# Autodesk Inventor assembly: pld-assembly
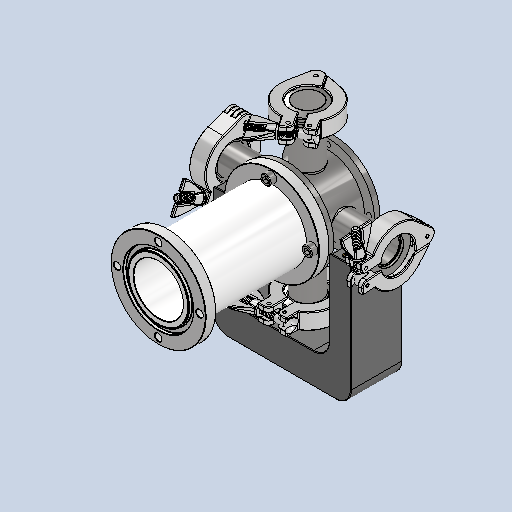
[picture p0: Inventor's stored thumbnail of the model, 512x512]
Saved by Autodesk Inventor 2026 (Build 300175050, 175E)
## iProperties
Created: 2025-11-13
Part Number: pld-assembly
Document SubType Name: Assembly
Designer: kuzmin
Author: kuzmin
## Documents named in this file (12)
- C:\Users\queez\Dropbox\Drawings\PIHTI\PLD\pld-assembly.iam
- C:\Users\queez\Dropbox\Drawings\PIHTI\PLD\pld-vessel-gasket.ipt
- C:\Users\queez\Dropbox\Drawings\PIHTI\ContentCenter\NW\NW25_clamp.ipt
- C:\Users\queez\Dropbox\Drawings\PIHTI\PLD\pld-vessel.iam
- C:\Users\queez\Dropbox\Drawings\PIHTI\PLD\pld_nipple.iam
- C:\Users\queez\Dropbox\Drawings\PIHTI\ContentCenter\Fastners\M6x16-SHCS.ipt
- C:\Users\queez\Dropbox\Drawings\PIHTI\PLD\pld-support.ipt
- C:\Users\queez\Dropbox\Drawings\PIHTI\ContentCenter\Fastners\brass-insert-m3x5.ipt
- C:\Users\queez\Dropbox\Drawings\PIHTI\ContentCenter\NW\NW25-blank.ipt
- C:\Users\queez\Dropbox\Drawings\PIHTI\PLD\pld-sample-holder.ipt
- C:\Users\queez\Dropbox\Drawings\PIHTI\PLD\m4x60-pin.ipt
- C:\Users\queez\Dropbox\Drawings\PIHTI\PLD\pld-target-holder.ipt
## Components (21 placed, 11 different names)
1. pld-vessel:1 [sub-assembly] — Rigid:7, Mate:2, Mate:3, Flush:2, Mate:5, Mate:6, Mate:7, Flush:3, Mate:8, Mate:9, Rigid:16, Rigid:18, Flush:4
2. pld-vessel-gasket:1
3. pld-vessel-gasket:2
4. NW25_clamp:1
5. pld_nipple:1 [sub-assembly] — Rigid:7, Rigid:8, Rigid:9, Rigid:10, Rigid:11
6. pld-support:1 — Mate:2, Mate:4, Rigid:12, Rigid:13, Rigid:14, Rigid:15, Mate:10
7. NW25_clamp:2 — Mate:5, Flush:3
8. NW25_clamp:3 — Mate:6, Mate:8
9. NW25_clamp:4 — Mate:7, Mate:9
10. brass-insert-m3x5:1 — Rigid:14
11. brass-insert-m3x5:2 — Rigid:13
12. brass-insert-m3x5:3 — Rigid:15
13. brass-insert-m3x5:4 — Rigid:12
14. NW25-blank:1 — Rigid:16, Rigid:17
15. pld-sample-holder:1 — Rotational:1
16. m4x60-pin:1 — Rigid:17, Rotational:1
17. pld-target-holder:1 — Rigid:18
18. JIS B 1176 - Metric M6 x 16:1 — Rigid:8
19. JIS B 1176 - Metric M6 x 16:2 — Rigid:9
20. JIS B 1176 - Metric M6 x 16:3 — Rigid:10
21. JIS B 1176 - Metric M6 x 16:4 — Rigid:11
## Relationships (29: WeldJoint 14, Mate 10, Flush 4, RevoluteJoint 1)
- [WeldJoint] (2 mm): pld-vessel:1 ↔ pld-vessel-gasket:1
- [WeldJoint] (2 mm): pld-vessel:1 ↔ pld-vessel-gasket:2
- [Mate]: pld-vessel:1 ↔ NW25_clamp:1
- [Flush]: pld-vessel:1 ↔ NW25_clamp:1
- Rigid:7 [WeldJoint]: pld-vessel:1 ↔ pld_nipple:1
- Rigid:8 [WeldJoint]: pld_nipple:1 ↔ JIS B 1176 - Metric M6 x 16:1
- Rigid:9 [WeldJoint]: pld_nipple:1 ↔ JIS B 1176 - Metric M6 x 16:2
- Rigid:10 [WeldJoint]: pld_nipple:1 ↔ JIS B 1176 - Metric M6 x 16:3
- Rigid:11 [WeldJoint]: pld_nipple:1 ↔ JIS B 1176 - Metric M6 x 16:4
- Mate:2: pld-vessel:1 ↔ pld-support:1
- Mate:3: pld-vessel:1
- Flush:2: pld-vessel:1
- Mate:4: pld-support:1
- Mate:5: pld-vessel:1 ↔ NW25_clamp:2
- Mate:6: pld-vessel:1 ↔ NW25_clamp:3
- Mate:7: pld-vessel:1 ↔ NW25_clamp:4
- Flush:3: pld-vessel:1 ↔ NW25_clamp:2
- Mate:8: pld-vessel:1 ↔ NW25_clamp:3
- Mate:9: pld-vessel:1 ↔ NW25_clamp:4
- Rigid:12 [WeldJoint]: pld-support:1 ↔ brass-insert-m3x5:4
- Rigid:13 [WeldJoint]: pld-support:1 ↔ brass-insert-m3x5:2
- Rigid:14 [WeldJoint]: pld-support:1 ↔ brass-insert-m3x5:1
- Rigid:15 [WeldJoint]: pld-support:1 ↔ brass-insert-m3x5:3
- Rigid:16 [WeldJoint] (2 mm): pld-vessel:1 ↔ NW25-blank:1
- Rigid:17 [WeldJoint]: NW25-blank:1 ↔ m4x60-pin:1
- Rotational:1 [RevoluteJoint]: pld-sample-holder:1 ↔ m4x60-pin:1
- Rigid:18 [WeldJoint]: pld-vessel:1 ↔ pld-target-holder:1
- Flush:4: pld-vessel:1
- Mate:10: pld-support:1
